# Autodesk Inventor assembly: M - hook block V2
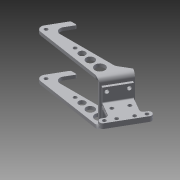
[picture p0: Inventor's stored thumbnail of the model, 180x180]
Saved by Autodesk Inventor 2013 (Build 170138000, 138)
## iProperties
Created: 2013-01-27
Part Number: M - hook block V2
Document SubType Name: Assembly
Designer: Arpan
Mass: 270.372 g
Surface Area: 484.572 cm^2
Volume: 99.7682 cm^3
Density: 2.71 g/cm^3
Author: Arpan
## Documents named in this file (9)
- C:\Users\Moses\Documents\GitHub\frc2013CAD\M-Climber\M - hook block V2.iam
- C:\Users\Moses\Documents\GitHub\frc2013CAD\M-Climber\M - Main Hook.ipt
- C:\Users\Moses\Documents\GitHub\frc2013CAD\M-Climber\M - Hook Mount Bracket.ipt
- C:\Users\Moses\Documents\GitHub\frc2013CAD\M-Climber\M - hook block V2\AIP\FEA\alrzqspts.fins
- C:\Users\Moses\Documents\GitHub\frc2013CAD\M-Climber\M - hook block V2\AIP\FEA\alrzqspts.fsat
- C:\Users\Moses\Documents\GitHub\frc2013CAD\M-Climber\M - hook block V2\AIP\FEA\alrzqspts.ftes
- C:\Users\Moses\Documents\GitHub\frc2013CAD\M-Climber\M - hook block V2\AIP\FEA\alrzqspts.fwiz
- C:\Users\Moses\Documents\GitHub\frc2013CAD\M-Climber\M - hook block V2\AIP\FEA\alrzqspuo.fmsh
- C:\Users\Moses\Documents\GitHub\frc2013CAD\M-Climber\M - hook block V2\AIP\FEA\als0fkgjk.fres
## Components (3 placed, 2 different names)
1. M - Main Hook:1 — Mate:1, Mate:2, Mate:3, Mate:4, Mate:5, Mate:6
2. M - Hook Mount Bracket:1 — Mate:1, Mate:2, Mate:3
3. M - Hook Mount Bracket:2 — Mate:4, Mate:5, Mate:6
## Relationships (6: Mate 6)
- Mate:1: M - Main Hook:1 ↔ M - Hook Mount Bracket:1
- Mate:2: M - Main Hook:1 ↔ M - Hook Mount Bracket:1
- Mate:3: M - Main Hook:1 ↔ M - Hook Mount Bracket:1
- Mate:4: M - Main Hook:1 ↔ M - Hook Mount Bracket:2
- Mate:5: M - Main Hook:1 ↔ M - Hook Mount Bracket:2
- Mate:6: M - Main Hook:1 ↔ M - Hook Mount Bracket:2
## Named parameters: sa_0 = -34574.7, sa_1 = 4.13685e-11, sa_2 = 81971.1
note: some values were not read from the file. Shown as the stored number, unit unknown: "sa_0", "sa_1", "sa_2".
